# Autodesk Inventor assembly: rearSwingarm
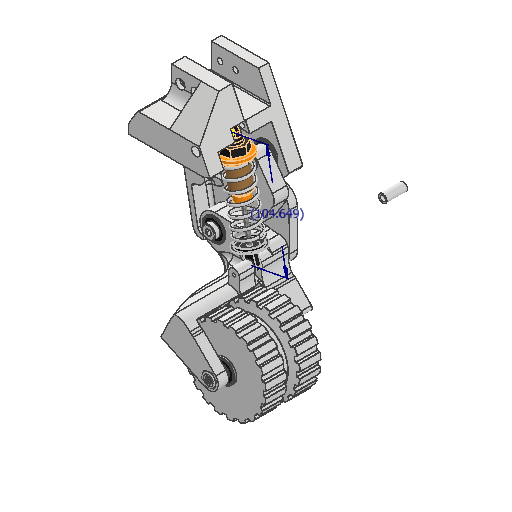
[picture p0: Inventor's stored thumbnail of the model, 512x512]
Saved by Autodesk Inventor 2025 (Build 290162000, 162)
## iProperties
Created: 2025-01-09
Part Number: rearSwingarm
Document SubType Name: Assembly
Designer: derm
Author: derm
## Documents named in this file (15)
- C:\Users\derm\Desktop\puppycat\rearSwingarm.iam
- C:\Users\derm\Desktop\puppycat\linkA.ipt
- C:\Users\derm\Desktop\puppycat\b link.ipt
- C:\Users\derm\Desktop\puppycat\printedWheel.ipt
- C:\Users\derm\Desktop\puppycat\linkC.ipt
- C:\Users\derm\Desktop\puppycat\6082rsBearing.ipt
- C:\Users\derm\Desktop\puppycat\swingarmBaseV5.ipt
- C:\Users\derm\Desktop\puppycat\100MMshockUpper.ipt
- C:\Users\derm\Desktop\puppycat\100MMshockLower.ipt
- C:\Users\derm\Desktop\puppycat\9002T445_Corrosion-Resistant Precision Compression Springs\9002T445_Corrosion-Resistant Precision Compression Springs.ipt
- C:\Users\derm\Desktop\puppycat\92981A203_Alloy Steel Shoulder Screws\92981A203_Alloy Steel Shoulder Screws.ipt
- C:\Users\derm\Desktop\puppycat\91290A461_Alloy Steel Socket Head Screw\91290A461_Alloy Steel Socket Head Screw.ipt
- C:\Users\derm\Desktop\puppycat\5mmAdapter.ipt
- C:\Users\derm\Desktop\puppycat\93070A175_Alloy Steel Low-Profile Socket Head Screw\93070A175_Alloy Steel Low-Profile Socket Head Screw.ipt
- C:\Users\derm\Desktop\puppycat\94645A210_High-Strength Steel Nylon-Insert Locknut\94645A210_High-Strength Steel Nylon-Insert Locknut.ipt
## Components (25 placed, 14 different names)
1. printedWheel:1 — Mate:23, Mate:24, Mate:41, Mate:43, Mate:44
2. 6082rsBearing:6 — Mate:24, Mate:41, Mate:52
3. swingarmBaseV5:1 — Mate:31, Mate:32, Mate:33, Mate:36, Mate:37, Mate:38, Mate:39, Mate:64, Mate:68
4. b link:2 — Mate:40, Mate:48, Mate:49, Mate:73, Mate:77, Mate:78, Mate:79, Mate:85, Mate:86, Angle:3
5. linkA:2 — Mate:34, Mate:35, Mate:46, Mate:47
6. linkC:2 — Mate:23, Mate:50, Mate:51, Mate:52, Mate:53, Mate:55, Mate:56, Mate:62, Mate:69, Mate:70, Mate:74, Mate:76, Mate:83, Angle:2, Mate:87
7. 6082rsBearing:7 — Mate:30, Mate:36, Mate:37
8. 6082rsBearing:8 — Mate:29, Mate:33
9. 6082rsBearing:9 — Mate:29, Mate:31, Mate:32, Mate:34, Mate:35
10. 6082rsBearing:10 — Mate:30, Mate:38, Mate:39, Mate:40, Mate:73
11. 6082rsBearing:11 — Mate:43, Mate:44
12. 6082rsBearing:12 — Mate:55, Mate:56, Flush:1, Mate:81, Mate:82
13. 6082rsBearing:14 — Mate:46, Mate:47, Mate:50, Mate:69
14. 6082rsBearing:15 — Mate:48, Mate:49, Mate:51, Mate:53, Mate:75
15. 100MMshockUpper:1 — Mate:64, Mate:68
16. 100MMshockLower:1 — Mate:70
17. 9002T445_Corrosion-Resistant Precision Compression Springs:1
18. 6082rsBearing:16 — Mate:62, Flush:1, Mate:74, Mate:75, Flush:2, Mate:80
19. 91290A461_Alloy Steel Socket Head Screw:1 — Mate:76
20. 92981A203_Alloy Steel Shoulder Screws:2 — Mate:77, Mate:78
21. 5mmAdapter:1 — Flush:2
22. 93070A175_Alloy Steel Low-Profile Socket Head Screw:1 — Mate:79, Mate:80
23. 93070A175_Alloy Steel Low-Profile Socket Head Screw:2 — Mate:81, Mate:82
24. 94645A210_High-Strength Steel Nylon-Insert Locknut:1 — Mate:83, Angle:2, Mate:87
25. 94645A210_High-Strength Steel Nylon-Insert Locknut:2 — Mate:85, Mate:86, Angle:3
## Relationships (54: Mate 49, Angle 3, Flush 2)
- Mate:23: printedWheel:1 ↔ linkC:2
- Mate:24: printedWheel:1 ↔ 6082rsBearing:6
- Mate:29: 6082rsBearing:8 ↔ 6082rsBearing:9
- Mate:30: 6082rsBearing:7 ↔ 6082rsBearing:10
- Mate:31: swingarmBaseV5:1 ↔ 6082rsBearing:9
- Mate:32: swingarmBaseV5:1 ↔ 6082rsBearing:9
- Mate:33: swingarmBaseV5:1 ↔ 6082rsBearing:8
- Mate:34: linkA:2 ↔ 6082rsBearing:9
- Mate:35: linkA:2 ↔ 6082rsBearing:9
- Mate:36: swingarmBaseV5:1 ↔ 6082rsBearing:7
- Mate:37: swingarmBaseV5:1 ↔ 6082rsBearing:7
- Mate:38: swingarmBaseV5:1 ↔ 6082rsBearing:10
- Mate:39: swingarmBaseV5:1 ↔ 6082rsBearing:10
- Mate:40: b link:2 ↔ 6082rsBearing:10
- Mate:41: printedWheel:1 ↔ 6082rsBearing:6
- Mate:43: printedWheel:1 ↔ 6082rsBearing:11
- Mate:44: printedWheel:1 ↔ 6082rsBearing:11
- Mate:46: linkA:2 ↔ 6082rsBearing:14
- Mate:47: linkA:2 ↔ 6082rsBearing:14
- Mate:48: b link:2 ↔ 6082rsBearing:15
- Mate:49: b link:2 ↔ 6082rsBearing:15
- Mate:50: linkC:2 ↔ 6082rsBearing:14
- Mate:51: linkC:2 ↔ 6082rsBearing:15
- Mate:52: 6082rsBearing:6 ↔ linkC:2
- Mate:53: linkC:2 ↔ 6082rsBearing:15
- Mate:55: linkC:2 ↔ 6082rsBearing:12
- Mate:56: linkC:2 ↔ 6082rsBearing:12
- [Mate]: 100MMshockUpper:1 ↔ 100MMshockLower:1
- [Angle] (0 deg): 100MMshockUpper:1 ↔ 100MMshockLower:1
- [Mate]: 100MMshockLower:1 ↔ 9002T445_Corrosion-Resistant Precision Compression Springs:1
- [Mate]: 100MMshockUpper:1 ↔ 9002T445_Corrosion-Resistant Precision Compression Springs:1
- Mate:62: linkC:2 ↔ 6082rsBearing:16
- Flush:1: 6082rsBearing:12 ↔ 6082rsBearing:16
- Mate:64 (20 mm): swingarmBaseV5:1 ↔ 100MMshockUpper:1
- Mate:68: swingarmBaseV5:1 ↔ 100MMshockUpper:1
- Mate:69: linkC:2 ↔ 6082rsBearing:14
- Mate:70: linkC:2 ↔ 100MMshockLower:1
- Mate:73: b link:2 ↔ 6082rsBearing:10
- Mate:74: linkC:2 ↔ 6082rsBearing:16
- Mate:75: 6082rsBearing:15 ↔ 6082rsBearing:16
- Mate:76: linkC:2 ↔ 91290A461_Alloy Steel Socket Head Screw:1
- Mate:77: b link:2 ↔ 92981A203_Alloy Steel Shoulder Screws:2
- Mate:78: b link:2 ↔ 92981A203_Alloy Steel Shoulder Screws:2
- Flush:2: 6082rsBearing:16 ↔ 5mmAdapter:1
- Mate:79: b link:2 ↔ 93070A175_Alloy Steel Low-Profile Socket Head Screw:1
- Mate:80: 6082rsBearing:16 ↔ 93070A175_Alloy Steel Low-Profile Socket Head Screw:1
- Mate:81: 6082rsBearing:12 ↔ 93070A175_Alloy Steel Low-Profile Socket Head Screw:2
- Mate:82: 6082rsBearing:12 ↔ 93070A175_Alloy Steel Low-Profile Socket Head Screw:2
- Mate:83: linkC:2 ↔ 94645A210_High-Strength Steel Nylon-Insert Locknut:1
- Angle:2 (0 deg): linkC:2 ↔ 94645A210_High-Strength Steel Nylon-Insert Locknut:1
- Mate:85: b link:2 ↔ 94645A210_High-Strength Steel Nylon-Insert Locknut:2
- Mate:86: b link:2 ↔ 94645A210_High-Strength Steel Nylon-Insert Locknut:2
- Angle:3 (0 deg): b link:2 ↔ 94645A210_High-Strength Steel Nylon-Insert Locknut:2
- Mate:87: linkC:2 ↔ 94645A210_High-Strength Steel Nylon-Insert Locknut:1
## Named parameters: d169_d73 = 0 mm, d170_d74 = 0 mm, d214_d0 = 0 mm, d215_d1 = 0 deg
